# Autodesk Inventor assembly: Sistema movimiento izquierdo
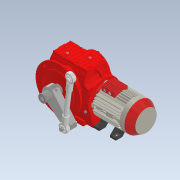
[picture p0: Inventor's stored thumbnail of the model, 180x180]
Saved by Autodesk Inventor 2021 (Build 250183000, 183)
## iProperties
Created: 2021-06-19
Part Number: Sistema movimiento izquierdo
Document SubType Name: Assembly
Designer: Andrés Holguín
Author: Andrés Holguín
## Documents named in this file (6)
- C:\Users\andre\Documents\GitHub\Dis.-Mecatronico-E6\inventor proyecto\Motores y reductores\Sistema movimiento izquierdo.iam
- C:\Users\andre\Documents\GitHub\Dis.-Mecatronico-E6\inventor proyecto\Motores y reductores\Reductor Izquierda.iam
- C:\Users\andre\Documents\GitHub\Dis.-Mecatronico-E6\inventor proyecto\Motores y reductores\placa manivela.ipt
- C:\Users\andre\Documents\GitHub\Dis.-Mecatronico-E6\inventor proyecto\Motores y reductores\pasador.ipt
- C:\Users\andre\Documents\GitHub\Dis.-Mecatronico-E6\inventor proyecto\Motores y reductores\Biela Completa.iam
- C:\Users\andre\Documents\GitHub\Dis.-Mecatronico-E6\inventor proyecto\Motores y reductores\Motor Simens Frame 112M IM B3.ipt
## Components (5 placed, 5 different names)
1. Reductor Izquierda:1 [sub-assembly] — Insert:3, Mate:1, Rigid:2
2. placa manivela:1 — Insert:3, Mate:1, Insert:4
3. pasador:1 — Insert:4, Insert:5
4. Motor Simens Frame 112M IM B3:1 — Rigid:2
5. Biela Completa:1 [sub-assembly] — Insert:5
## Relationships (5: Insert 3, Mate 1, WeldJoint 1)
- Insert:3 (50 mm): Reductor Izquierda:1 ↔ placa manivela:1
- Mate:1: Reductor Izquierda:1 ↔ placa manivela:1
- Insert:4: placa manivela:1 ↔ pasador:1
- Rigid:2 [WeldJoint]: Reductor Izquierda:1 ↔ Motor Simens Frame 112M IM B3:1
- Insert:5 (15 mm): pasador:1 ↔ Biela Completa:1
